# Autodesk Inventor assembly: TPS
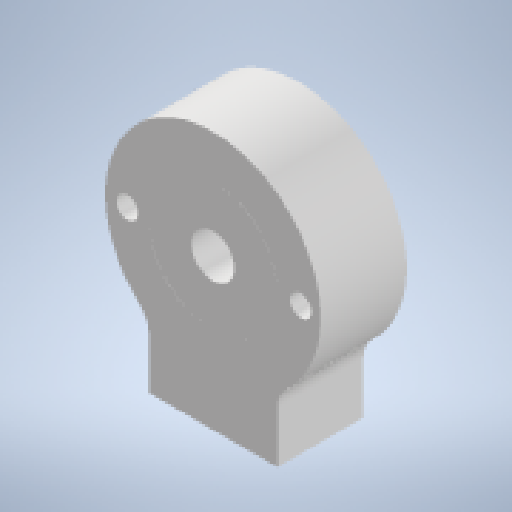
[picture p0: Inventor's stored thumbnail of the model, 512x512]
Saved by Autodesk Inventor 2023 (Build 270158000, 158)
## iProperties
Created: 2023-07-25
Part Number: TPS
Document SubType Name: Assembly
Designer: User
Author: User
## Documents named in this file (3)
- C:\Users\User\Desktop\BIANCA\SCHOOL WORK\INVENTOR 2023\CRUISE CONTROL\TPS.iam
- C:\Users\User\Desktop\BIANCA\SCHOOL WORK\INVENTOR 2023\CRUISE CONTROL\TPS base.ipt
- C:\Users\User\Desktop\BIANCA\SCHOOL WORK\INVENTOR 2023\CRUISE CONTROL\TPS inner.ipt
## Components (2 placed, 2 different names)
1. TPS base:1 — Insert:1
2. TPS inner:1 — Insert:1
## Relationships (1: Insert 1)
- Insert:1: TPS base:1 ↔ TPS inner:1
